# Autodesk Inventor assembly: Keeyboard_Assemply
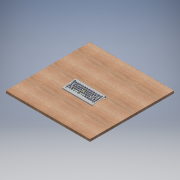
[picture p0: Inventor's stored thumbnail of the model, 180x180]
Saved by Autodesk Inventor 2018 (Build 220112000, 112)
## iProperties
Created: 2018-02-08
Part Number: Keeyboard_Assemply
Document SubType Name: Assembly
Designer: ConnorDevitt
Author: ConnorDevitt
## Documents named in this file (8)
- C:\Users\ConnorDevitt.MSI\Documents\Keyboard\60pc_Keeb\HW\3D\Keeyboard_Assemply.iam
- C:\Users\ConnorDevitt.MSI\Documents\Keyboard\60pc_Keeb\HW\3D\Frame.ipt
- C:\Users\ConnorDevitt.MSI\Documents\Keyboard\60pc_Keeb\HW\3D\Desk.ipt
- C:\Users\ConnorDevitt.MSI\Documents\Keyboard\60pc_Keeb\HW\3D\60pc_pcb.kicad_pcb_Outline.ipt
- C:\Users\ConnorDevitt.MSI\Documents\Keyboard\60pc_Keeb\HW\3D\User Library-USB-Mini-B.ipt
- C:\Users\ConnorDevitt.MSI\Documents\Keyboard\60pc_Keeb\HW\3D\MX .ipt
- C:\Users\ConnorDevitt.MSI\Documents\Keyboard\60pc_Keeb\HW\3D\Stabilizer - close.ipt
- C:\Users\ConnorDevitt.MSI\Documents\Inventor\Content Center Files\R2018\en-US\ISO 7046-1(1)\DIN EN ISO 7046-1 - M4 x 12 - 4.8 - H.ipt
## Components (79 placed, 7 different names)
1. Desk:1 — Rigid:71
2. 60pc_pcb.kicad_pcb_Outline:1 — Rigid:2, Rigid:3, Rigid:4, Rigid:5, Rigid:6, Rigid:7, Rigid:8, Rigid:9, Rigid:10, Rigid:11, Rigid:12, Rigid:13, Rigid:14, Rigid:15, Rigid:16, Rigid:17, Rigid:18, Rigid:19, Rigid:20, Rigid:21, Rigid:22, Rigid:23, Rigid:24, Rigid:25, Rigid:26, Rigid:27, Rigid:28, Rigid:29, Rigid:30, Rigid:31, Rigid:32, Rigid:33, Rigid:34, Rigid:35, Rigid:36, Rotational:5, Rigid:37, Rigid:38, Rigid:39, Rigid:40, Rigid:41, Rigid:42, Rigid:43, Rigid:44, Rigid:45, Rigid:46, Rigid:47, Rigid:48, Rigid:49, Rigid:50, Rigid:51, Rigid:52, Rigid:53, Rigid:54, Rigid:55, Rigid:56, Rigid:57, Rigid:58, Rigid:59, Rigid:60, Rigid:61, Rigid:62, Rigid:63, Rigid:64, Rigid:65, Rigid:66, Rigid:67, Rigid:68, Rigid:69, Rigid:70, Rigid:72, Rigid:73, Rigid:74
3. MX :1 — Rigid:68
4. MX :2 — Rigid:40
5. MX :3 — Rigid:69
6. MX :4 — Rigid:37
7. MX :5 — Rigid:19
8. MX :6 — Rigid:34
9. MX :7 — Rigid:59
10. MX :8 — Rigid:31
11. MX :9 — Rigid:17
12. MX :10 — Rigid:16
13. MX :11 — Rigid:47
14. MX :12 — Rigid:48
15. MX :13 — Rigid:54
16. MX :14 — Rigid:52
17. MX :15 — Rigid:44
18. MX :16 — Rigid:32
19. MX :17 — Rigid:46
20. MX :18 — Rigid:49
21. MX :19 — Rigid:57
22. MX :20 — Rigid:56
23. MX :21 — Rigid:35
24. MX :22 — Rigid:53
25. MX :23 — Rigid:28
26. MX :24 — Rigid:15
27. MX :25 — Rigid:18
28. MX :26 — Rigid:70
29. MX :27 — Rigid:67
30. MX :28 — Rigid:29
31. MX :29 — Rigid:51
32. MX :30 — Rigid:14
33. MX :31 — Rotational:5
34. MX :32 — Rigid:33
35. MX :33 — Rigid:61
36. MX :34 — Rigid:63
37. MX :35 — Rigid:39
38. MX :36 — Rigid:38
39. MX :37 — Rigid:64
40. MX :38 — Rigid:66
41. MX :39 — Rigid:30
42. MX :40 — Rigid:36
43. MX :41 — Rigid:62
44. MX :42 — Rigid:42
45. MX :43 — Rigid:50
46. MX :44 — Rigid:45
47. MX :45 — Rigid:43
48. MX :46 — Rigid:65
49. MX :47 — Rigid:60
50. MX :48 — Rigid:58
51. MX :49 — Rigid:55
52. MX :50 — Rigid:41
53. MX :51 — Rigid:20
54. MX :55 — Rigid:6
55. MX :56 — Rigid:5
56. MX :57 — Rigid:8
57. MX :58 — Rigid:23
58. MX :59 — Rigid:26
59. MX :60 — Rigid:24
60. MX :61 — Rigid:21
61. MX :62 — Rigid:27
62. MX :63 — Rigid:11
63. MX :64 — Rigid:4
64. MX :65 — Rigid:13
65. MX :66 — Rigid:22
66. MX :67 — Rigid:9
67. MX :69 — Rigid:7
68. MX :70 — Rigid:25
69. MX :71 — Rigid:12
70. MX :72 — Rigid:10
71. Stabilizer - close:1 — Rigid:72
72. Stabilizer - close:2 — Rigid:74
73. Stabilizer - close:3 — Rigid:73
74. Frame:1 — Rigid:2, Rotational:1, Rotational:2, Rotational:3, Rotational:4, Rigid:71
75. DIN EN ISO 7046-1 H M4 x 12 - 4.8 - H:2 — Rotational:2
76. DIN EN ISO 7046-1 H M4 x 12 - 4.8 - H:3 — Rotational:4
77. DIN EN ISO 7046-1 H M4 x 12 - 4.8 - H:4 — Rotational:3
78. DIN EN ISO 7046-1 H M4 x 12 - 4.8 - H:5 — Rotational:1
79. User Library-USB-Mini-B:2 — Rigid:3
## Relationships (78: WeldJoint 73, RevoluteJoint 5)
- Rigid:2 [WeldJoint] (-2.3876 mm): 60pc_pcb.kicad_pcb_Outline:1 ↔ Frame:1
- Rotational:1 [RevoluteJoint]: Frame:1 ↔ DIN EN ISO 7046-1 H M4 x 12 - 4.8 - H:5
- Rotational:2 [RevoluteJoint]: Frame:1 ↔ DIN EN ISO 7046-1 H M4 x 12 - 4.8 - H:2
- Rotational:3 [RevoluteJoint]: Frame:1 ↔ DIN EN ISO 7046-1 H M4 x 12 - 4.8 - H:4
- Rotational:4 [RevoluteJoint]: Frame:1 ↔ DIN EN ISO 7046-1 H M4 x 12 - 4.8 - H:3
- Rigid:3 [WeldJoint]: 60pc_pcb.kicad_pcb_Outline:1 ↔ User Library-USB-Mini-B:2
- Rigid:4 [WeldJoint]: 60pc_pcb.kicad_pcb_Outline:1 ↔ MX :64
- Rigid:5 [WeldJoint]: 60pc_pcb.kicad_pcb_Outline:1 ↔ MX :56
- Rigid:6 [WeldJoint]: 60pc_pcb.kicad_pcb_Outline:1 ↔ MX :55
- Rigid:7 [WeldJoint]: 60pc_pcb.kicad_pcb_Outline:1 ↔ MX :69
- Rigid:8 [WeldJoint]: 60pc_pcb.kicad_pcb_Outline:1 ↔ MX :57
- Rigid:9 [WeldJoint]: 60pc_pcb.kicad_pcb_Outline:1 ↔ MX :67
- Rigid:10 [WeldJoint]: 60pc_pcb.kicad_pcb_Outline:1 ↔ MX :72
- Rigid:11 [WeldJoint]: 60pc_pcb.kicad_pcb_Outline:1 ↔ MX :63
- Rigid:12 [WeldJoint]: 60pc_pcb.kicad_pcb_Outline:1 ↔ MX :71
- Rigid:13 [WeldJoint]: 60pc_pcb.kicad_pcb_Outline:1 ↔ MX :65
- Rigid:14 [WeldJoint]: 60pc_pcb.kicad_pcb_Outline:1 ↔ MX :30
- Rigid:15 [WeldJoint]: 60pc_pcb.kicad_pcb_Outline:1 ↔ MX :24
- Rigid:16 [WeldJoint]: 60pc_pcb.kicad_pcb_Outline:1 ↔ MX :10
- Rigid:17 [WeldJoint]: 60pc_pcb.kicad_pcb_Outline:1 ↔ MX :9
- Rigid:18 [WeldJoint]: 60pc_pcb.kicad_pcb_Outline:1 ↔ MX :25
- Rigid:19 [WeldJoint]: 60pc_pcb.kicad_pcb_Outline:1 ↔ MX :5
- Rigid:20 [WeldJoint]: 60pc_pcb.kicad_pcb_Outline:1 ↔ MX :51
- Rigid:21 [WeldJoint]: 60pc_pcb.kicad_pcb_Outline:1 ↔ MX :61
- Rigid:22 [WeldJoint]: 60pc_pcb.kicad_pcb_Outline:1 ↔ MX :66
- Rigid:23 [WeldJoint]: 60pc_pcb.kicad_pcb_Outline:1 ↔ MX :58
- Rigid:24 [WeldJoint]: 60pc_pcb.kicad_pcb_Outline:1 ↔ MX :60
- Rigid:25 [WeldJoint]: 60pc_pcb.kicad_pcb_Outline:1 ↔ MX :70
- Rigid:26 [WeldJoint]: 60pc_pcb.kicad_pcb_Outline:1 ↔ MX :59
- Rigid:27 [WeldJoint]: 60pc_pcb.kicad_pcb_Outline:1 ↔ MX :62
- Rigid:28 [WeldJoint]: 60pc_pcb.kicad_pcb_Outline:1 ↔ MX :23
- Rigid:29 [WeldJoint]: 60pc_pcb.kicad_pcb_Outline:1 ↔ MX :28
- Rigid:30 [WeldJoint]: 60pc_pcb.kicad_pcb_Outline:1 ↔ MX :39
- Rigid:31 [WeldJoint]: 60pc_pcb.kicad_pcb_Outline:1 ↔ MX :8
- Rigid:32 [WeldJoint]: 60pc_pcb.kicad_pcb_Outline:1 ↔ MX :16
- Rigid:33 [WeldJoint]: 60pc_pcb.kicad_pcb_Outline:1 ↔ MX :32
- Rigid:34 [WeldJoint]: 60pc_pcb.kicad_pcb_Outline:1 ↔ MX :6
- Rigid:35 [WeldJoint]: 60pc_pcb.kicad_pcb_Outline:1 ↔ MX :21
- Rigid:36 [WeldJoint]: 60pc_pcb.kicad_pcb_Outline:1 ↔ MX :40
- Rotational:5 [RevoluteJoint]: 60pc_pcb.kicad_pcb_Outline:1 ↔ MX :31
- Rigid:37 [WeldJoint]: 60pc_pcb.kicad_pcb_Outline:1 ↔ MX :4
- Rigid:38 [WeldJoint]: 60pc_pcb.kicad_pcb_Outline:1 ↔ MX :36
- Rigid:39 [WeldJoint]: 60pc_pcb.kicad_pcb_Outline:1 ↔ MX :35
- Rigid:40 [WeldJoint]: 60pc_pcb.kicad_pcb_Outline:1 ↔ MX :2
- Rigid:41 [WeldJoint]: 60pc_pcb.kicad_pcb_Outline:1 ↔ MX :50
- Rigid:42 [WeldJoint]: 60pc_pcb.kicad_pcb_Outline:1 ↔ MX :42
- Rigid:43 [WeldJoint]: 60pc_pcb.kicad_pcb_Outline:1 ↔ MX :45
- Rigid:44 [WeldJoint]: 60pc_pcb.kicad_pcb_Outline:1 ↔ MX :15
- Rigid:45 [WeldJoint]: 60pc_pcb.kicad_pcb_Outline:1 ↔ MX :44
- Rigid:46 [WeldJoint]: 60pc_pcb.kicad_pcb_Outline:1 ↔ MX :17
- Rigid:47 [WeldJoint]: 60pc_pcb.kicad_pcb_Outline:1 ↔ MX :11
- Rigid:48 [WeldJoint]: 60pc_pcb.kicad_pcb_Outline:1 ↔ MX :12
- Rigid:49 [WeldJoint]: 60pc_pcb.kicad_pcb_Outline:1 ↔ MX :18
- Rigid:50 [WeldJoint]: 60pc_pcb.kicad_pcb_Outline:1 ↔ MX :43
- Rigid:51 [WeldJoint]: 60pc_pcb.kicad_pcb_Outline:1 ↔ MX :29
- Rigid:52 [WeldJoint]: 60pc_pcb.kicad_pcb_Outline:1 ↔ MX :14
- Rigid:53 [WeldJoint]: 60pc_pcb.kicad_pcb_Outline:1 ↔ MX :22
- Rigid:54 [WeldJoint]: 60pc_pcb.kicad_pcb_Outline:1 ↔ MX :13
- Rigid:55 [WeldJoint]: 60pc_pcb.kicad_pcb_Outline:1 ↔ MX :49
- Rigid:56 [WeldJoint]: 60pc_pcb.kicad_pcb_Outline:1 ↔ MX :20
- Rigid:57 [WeldJoint]: 60pc_pcb.kicad_pcb_Outline:1 ↔ MX :19
- Rigid:58 [WeldJoint]: 60pc_pcb.kicad_pcb_Outline:1 ↔ MX :48
- Rigid:59 [WeldJoint]: 60pc_pcb.kicad_pcb_Outline:1 ↔ MX :7
- Rigid:60 [WeldJoint]: 60pc_pcb.kicad_pcb_Outline:1 ↔ MX :47
- Rigid:61 [WeldJoint]: 60pc_pcb.kicad_pcb_Outline:1 ↔ MX :33
- Rigid:62 [WeldJoint]: 60pc_pcb.kicad_pcb_Outline:1 ↔ MX :41
- Rigid:63 [WeldJoint]: 60pc_pcb.kicad_pcb_Outline:1 ↔ MX :34
- Rigid:64 [WeldJoint]: 60pc_pcb.kicad_pcb_Outline:1 ↔ MX :37
- Rigid:65 [WeldJoint]: 60pc_pcb.kicad_pcb_Outline:1 ↔ MX :46
- Rigid:66 [WeldJoint]: 60pc_pcb.kicad_pcb_Outline:1 ↔ MX :38
- Rigid:67 [WeldJoint]: 60pc_pcb.kicad_pcb_Outline:1 ↔ MX :27
- Rigid:68 [WeldJoint]: 60pc_pcb.kicad_pcb_Outline:1 ↔ MX :1
- Rigid:69 [WeldJoint]: 60pc_pcb.kicad_pcb_Outline:1 ↔ MX :3
- Rigid:70 [WeldJoint]: 60pc_pcb.kicad_pcb_Outline:1 ↔ MX :26
- Rigid:72 [WeldJoint]: 60pc_pcb.kicad_pcb_Outline:1 ↔ Stabilizer - close:1
- Rigid:73 [WeldJoint]: 60pc_pcb.kicad_pcb_Outline:1 ↔ Stabilizer - close:3
- Rigid:74 [WeldJoint]: 60pc_pcb.kicad_pcb_Outline:1 ↔ Stabilizer - close:2
- Rigid:71 [WeldJoint]: Desk:1 ↔ Frame:1
